# Autodesk Inventor assembly: ведро с круто
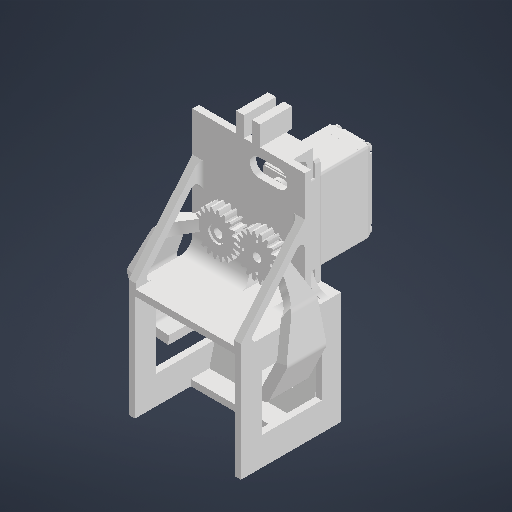
[picture p0: Inventor's stored thumbnail of the model, 512x512]
Saved by Autodesk Inventor 2025 (Build 290162000, 162)
## iProperties
Created: 2025-01-15
Part Number: ведро с круто
Document SubType Name: Assembly
Designer: Phantom
Author: Phantom
## Documents named in this file (5)
- C:\Users\Phantom\Desktop\Phantom16950\ведро с круто.iam
- C:\Users\Phantom\Desktop\Phantom16950\ведро.ipt
- C:\Users\Phantom\Desktop\Phantom16950\манипулятор 1.ipt
- C:\Users\Phantom\Desktop\Phantom16950\2000-0025-0002\2000-0025-0002.ipt
- C:\Users\Phantom\Desktop\Phantom16950\манипулятор 2.ipt
## Components (4 placed, 4 different names)
1. ведро:1 — Совмещение:1, Заподлицо:1, Совмещение:3, Совмещение:4, Совмещение:5
2. манипулятор 1:1 — Совмещение:4, Совмещение:5
3. 2000-0025-0002:1 — Совмещение:1, Заподлицо:1, Совмещение:2
4. манипулятор 2:1 — Совмещение:2, Совмещение:3
## Relationships (6: Mate 5, Flush 1)
- Совмещение:1 [Mate]: ведро:1 ↔ 2000-0025-0002:1
- Заподлицо:1 [Flush] (-1 mm): ведро:1 ↔ 2000-0025-0002:1
- Совмещение:2 [Mate]: 2000-0025-0002:1 ↔ манипулятор 2:1
- Совмещение:3 [Mate]: ведро:1 ↔ манипулятор 2:1
- Совмещение:4 [Mate]: ведро:1 ↔ манипулятор 1:1
- Совмещение:5 [Mate]: ведро:1 ↔ манипулятор 1:1
